# Autodesk Inventor assembly: 4-7
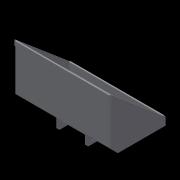
[picture p0: Inventor's stored thumbnail of the model, 180x180]
Saved by Autodesk Inventor 2017 (Build 210142000, 142)
## iProperties
Part Number: 4-7
Material: 一般
Document SubType Name: Assembly
Designer: r0909
Author: r0909
## Documents named in this file (5)
- C:\Users\r0909\Desktop\inventor\4-7.iam
- C:\Users\r0909\Desktop\inventor\4-4.ipt
- C:\Users\r0909\Desktop\inventor\4-5.ipt
- C:\Users\r0909\Desktop\inventor\4-6a.ipt
- C:\Users\r0909\Desktop\inventor\4-6b.ipt
## Components (4 placed, 4 different names)
1. 4-4:1 — 貼合:7, 貼合:8, 貼合:9
2. 4-5:1 — 貼合:1, 貼合:2, 貼合:3, 貼合:4, 貼合:5, 貼合:6, 貼合:7, 貼合:8, 貼合:9
3. 4-6a:1 — 貼合:1, 貼合:2, 貼合:3
4. 4-6b:1 — 貼合:4, 貼合:5, 貼合:6
## Relationships (9: Mate 9)
- 貼合:1 [Mate]: 4-5:1 ↔ 4-6a:1
- 貼合:2 [Mate]: 4-5:1 ↔ 4-6a:1
- 貼合:3 [Mate]: 4-5:1 ↔ 4-6a:1
- 貼合:4 [Mate]: 4-5:1 ↔ 4-6b:1
- 貼合:5 [Mate]: 4-5:1 ↔ 4-6b:1
- 貼合:6 [Mate]: 4-5:1 ↔ 4-6b:1
- 貼合:7 [Mate]: 4-4:1 ↔ 4-5:1
- 貼合:8 [Mate]: 4-4:1 ↔ 4-5:1
- 貼合:9 [Mate]: 4-4:1 ↔ 4-5:1
